# Autodesk Inventor assembly: Ensamblaje del tambor con sis. Lebus - V1
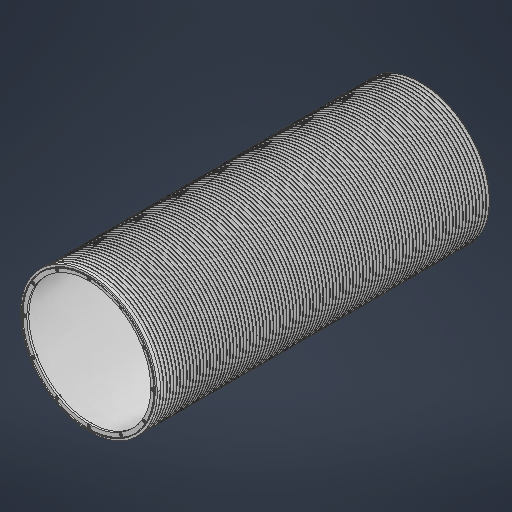
[picture p0: Inventor's stored thumbnail of the model, 512x512]
Saved by Autodesk Inventor 2026 (Build 300175050, 175E)
## iProperties
Created: 2025-07-12
Part Number: Ensamblaje del tambor con sis. Lebus - V1
Document SubType Name: Assembly
Designer: Daniel Rodriguez
Author: Daniel Rodriguez
## Documents named in this file (5)
- C:\Users\Daniel Rodriguez\Downloads\winch-drum-welding-assembly\Nuestro Winch\Sistema LEBUS\Ensamblaje del tambor con sis. Lebus - V1.iam
- C:\Users\Daniel Rodriguez\Downloads\winch-drum-welding-assembly\Nuestro Winch\Sistema LEBUS\Tambor liso (drum).ipt
- C:\Users\Daniel Rodriguez\Downloads\winch-drum-welding-assembly\Nuestro Winch\Sistema LEBUS\Sistema LEBUS.ipt
- C:\Users\Daniel Rodriguez\Downloads\winch-drum-welding-assembly\Nuestro Winch\Sistema LEBUS\Aro del tambor.ipt
- C:\Users\Daniel Rodriguez\Downloads\winch-drum-welding-assembly\Nuestro Winch\Sistema LEBUS\95105A199_Zinc-Plated Steel Heavy-Duty Rivet Nut.ipt
## Components (28 placed, 4 different names)
1. Tambor liso (drum):1 — Insertar:1, Insertar:2, Insertar:3
2. Sistema LEBUS:1 — Insertar:1
3. Aro del tambor:1 — Insertar:2, Insertar:4
4. Aro del tambor:2 — Insertar:3, Insertar:5
5. 95105A199_Zinc-Plated Steel Heavy-Duty Rivet Nut:1 — Insertar:4
6. 95105A199_Zinc-Plated Steel Heavy-Duty Rivet Nut:2
7. 95105A199_Zinc-Plated Steel Heavy-Duty Rivet Nut:3
8. 95105A199_Zinc-Plated Steel Heavy-Duty Rivet Nut:4
9. 95105A199_Zinc-Plated Steel Heavy-Duty Rivet Nut:5
10. 95105A199_Zinc-Plated Steel Heavy-Duty Rivet Nut:6
11. 95105A199_Zinc-Plated Steel Heavy-Duty Rivet Nut:7
12. 95105A199_Zinc-Plated Steel Heavy-Duty Rivet Nut:8
13. 95105A199_Zinc-Plated Steel Heavy-Duty Rivet Nut:9
14. 95105A199_Zinc-Plated Steel Heavy-Duty Rivet Nut:10
15. 95105A199_Zinc-Plated Steel Heavy-Duty Rivet Nut:11
16. 95105A199_Zinc-Plated Steel Heavy-Duty Rivet Nut:12
17. 95105A199_Zinc-Plated Steel Heavy-Duty Rivet Nut:13 — Insertar:5
18. 95105A199_Zinc-Plated Steel Heavy-Duty Rivet Nut:14
19. 95105A199_Zinc-Plated Steel Heavy-Duty Rivet Nut:15
20. 95105A199_Zinc-Plated Steel Heavy-Duty Rivet Nut:16
21. 95105A199_Zinc-Plated Steel Heavy-Duty Rivet Nut:17
22. 95105A199_Zinc-Plated Steel Heavy-Duty Rivet Nut:18
23. 95105A199_Zinc-Plated Steel Heavy-Duty Rivet Nut:19
24. 95105A199_Zinc-Plated Steel Heavy-Duty Rivet Nut:20
25. 95105A199_Zinc-Plated Steel Heavy-Duty Rivet Nut:21
26. 95105A199_Zinc-Plated Steel Heavy-Duty Rivet Nut:22
27. 95105A199_Zinc-Plated Steel Heavy-Duty Rivet Nut:23
28. 95105A199_Zinc-Plated Steel Heavy-Duty Rivet Nut:24
## Component patterns: (12 elements, first: 95105A199_Zinc-Plated Steel Heavy-Duty Rivet Nut:1), (12 elements, first: 95105A199_Zinc-Plated Steel Heavy-Duty Rivet Nut:13)
## Relationships (5: Insert 5)
- Insertar:1 (5 mm): Tambor liso (drum):1 ↔ Sistema LEBUS:1
- Insertar:2 (5 mm): Tambor liso (drum):1 ↔ Aro del tambor:1
- Insertar:3 (5 mm): Tambor liso (drum):1 ↔ Aro del tambor:2
- Insertar:4: Aro del tambor:1 ↔ 95105A199_Zinc-Plated Steel Heavy-Duty Rivet Nut:1
- Insertar:5: Aro del tambor:2 ↔ 95105A199_Zinc-Plated Steel Heavy-Duty Rivet Nut:13
